# Autodesk Inventor assembly: SSR-on-DIN-mount
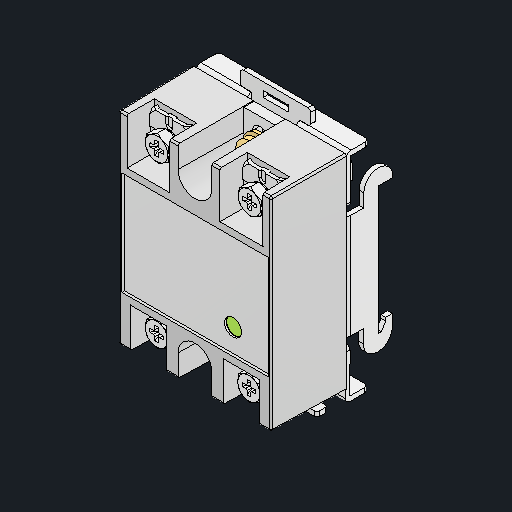
[picture p0: Inventor's stored thumbnail of the model, 512x512]
Saved by Autodesk Inventor 2027.1 (Build 311270010, 270A)
## iProperties
Created: 2025-06-05
Part Number: SSR-on-DIN-mount
Document SubType Name: Assembly
Designer: queezz
Author: queezz
## Documents named in this file (3)
- C:\Users\queezz\Dropbox\Drawings\PIHTI\ElectronicsBox\TempController-v2\SSR-on-DIN-mount.iam
- C:\Users\queezz\Dropbox\Drawings\PIHTI\ElectronicsBox\TempController\Solid State Relay\Solid State Relay backp.iam
- C:\Users\queezz\Dropbox\Drawings\PIHTI\ElectronicsBox\TempController\SSR Din Rail Mount\SSR Din Rail Mount.iam
## Components (2 placed, 2 different names)
1. Solid State Relay backp:1 [sub-assembly]
2. SSR Din Rail Mount:1 [sub-assembly]
## Relationships (2: Mate 2)
- [Mate]: Solid State Relay backp:1 ↔ SSR Din Rail Mount:1
- [Mate]: Solid State Relay backp:1 ↔ SSR Din Rail Mount:1
